# Autodesk Inventor assembly: sestava tělo estonsko s plechem otočené motory
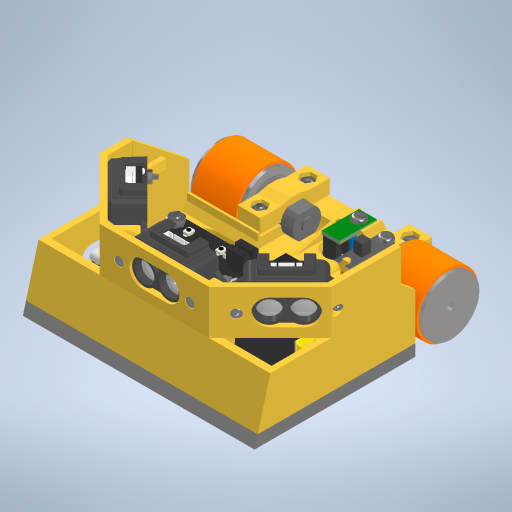
[picture p0: Inventor's stored thumbnail of the model, 512x512]
Saved by Autodesk Inventor 2024 (Build 280153000, 153)
## iProperties
Created: 2023-11-14
Part Number: sestava tělo estonsko s plechem otočené motory
Document SubType Name: Assembly
Designer: Simak
Author: Simak
## Documents named in this file (22)
- C:\Users\Simak\OneDrive\Dokumenty\GitHub\RoboCop\- 3D -\archive\body_v3.0_(Estonsko)\Tělo s plechem\sestava tělo estonsko s plechem otočené motory.iam
- C:\Users\Simak\OneDrive\Dokumenty\GitHub\RoboCop\- 3D -\archive\body_v3.0_(Estonsko)\Tělo s plechem\tělo estonsko s plechem otočené motory.ipt
- C:\Users\Simak\OneDrive\Dokumenty\GitHub\RoboCop\- 3D -\mech._parts\plech.ipt
- C:\Users\Simak\OneDrive\Dokumenty\GitHub\RoboCop\- 3D -\el._parts\sumec_smd.iam
- C:\Users\Simak\OneDrive\Dokumenty\GitHub\RoboCop\- 3D -\archive\TF-Luna_holder_v1\Sestava TF-Luna a držáku.iam
- C:\Users\Simak\OneDrive\Dokumenty\GitHub\RoboCop\- 3D -\el._parts\qre_module.ipt
- C:\Users\Simak\OneDrive\Dokumenty\GitHub\RoboCop\- 3D -\el._parts\switch.ipt
- C:\Users\Simak\OneDrive\Dokumenty\GitHub\RoboCop\- 3D -\el._parts\GA12-N20_Motor.ipt
- C:\Users\Simak\OneDrive\Dokumenty\GitHub\RoboCop\- 3D -\mech._parts\wheel+silicon.ipt
- C:\Users\Simak\OneDrive\Dokumenty\GitHub\RoboCop\- 3D -\mech._parts\motor_C_clamp_nutt_motor_otoceny.ipt
- C:\Users\Simak\OneDrive\Dokumenty\GitHub\RoboCop\- 3D -\screws+nuts\screws\M3_kuzel_torx\torx_socket_countersunk_flat_head_M3x18.ipt
- C:\Users\Simak\OneDrive\Dokumenty\GitHub\RoboCop\- 3D -\screws+nuts\nuts\M3 Nut.ipt
- C:\Users\Simak\OneDrive\Dokumenty\GitHub\RoboCop\- 3D -\screws+nuts\screws\M3_kuzel_torx\torx_socket_countersunk_flat_head_M3x08.ipt
- C:\Users\Simak\OneDrive\Dokumenty\GitHub\RoboCop\- 3D -\screws+nuts\screws\M3_koule_torx\torx_socket_button_head_M3x08.ipt
- C:\Users\Simak\OneDrive\Dokumenty\GitHub\RoboCop\- 3D -\screws+nuts\screws\M3_kuzel_torx\torx_socket_countersunk_flat_head_M3x12.ipt
- C:\Users\Simak\OneDrive\Dokumenty\GitHub\RoboCop\- 3D -\screws+nuts\screws\M3_koule_torx\torx_socket_button_head_M3x10.ipt
- C:\Users\Simak\OneDrive\Dokumenty\GitHub\RoboCop\- 3D -\screws+nuts\screws\M2_valec_imbus\M2 x 0.4mm Thread 16mm LONG SOCKET HEAD CAP SCREW.ipt
- C:\Users\Simak\OneDrive\Dokumenty\GitHub\RoboCop\- 3D -\screws+nuts\screws\M2_valec_imbus\M2 x 0.4mm Thread 12mm LONG SOCKET HEAD CAP SCREW.ipt
- C:\Users\Simak\OneDrive\Dokumenty\GitHub\RoboCop\- 3D -\el._parts\connectors\XT30\XT30_Stecker.ipt
- C:\Users\Simak\OneDrive\Dokumenty\GitHub\RoboCop\- 3D -\screws+nuts\nuts\M2 x 0.4mm Thread HEX NUT.ipt
- C:\Users\Simak\OneDrive\Dokumenty\GitHub\RoboCop\- 3D -\mech._parts\oddělovací plocha.ipt
- C:\Users\Simak\OneDrive\Dokumenty\GitHub\RoboCop\- 3D -\archive\body_v3.0_(Estonsko)\Tělo s plechem\kryt.ipt
## Components (51 placed, 21 different names)
1. tělo estonsko s plechem otočené motory:1 — Proti sobě:1, Stejný směr:1, Stejný směr:2, Proti sobě:2, Vložit:1, Vložit:2, Proti sobě:3, Proti sobě:4, Stejný směr:3, Vložit:3, Proti sobě:5, Proti sobě:6, Proti sobě:7, Proti sobě:8, Proti sobě:10, Proti sobě:11, Proti sobě:12, Proti sobě:13, Proti sobě:14, Proti sobě:15, Stejný směr:4, Stejný směr:5, Proti sobě:19, Vložit:4, Proti sobě:21, Vložit:5, Vložit:8, Vložit:9, Proti sobě:28, Proti sobě:39, Proti sobě:40, Vložit:27, Vložit:28, Proti sobě:41, Proti sobě:42, Vložit:34, Proti sobě:45, Proti sobě:47, Proti sobě:48, Proti sobě:49, Stejný směr:6
2. plech:1 — Proti sobě:1, Stejný směr:1, Stejný směr:2, Vložit:6, Vložit:7, Vložit:11, Vložit:12, Vložit:13, Vložit:14, Proti sobě:46, Vložit:35
3. sumec_smd:1 [sub-assembly] — Proti sobě:2, Vložit:1, Vložit:2, Proti sobě:34, Proti sobě:35, Proti sobě:36, Vložit:23, Vložit:24, Vložit:25, Vložit:26
4. Sestava TF-Luna a držáku:1 [sub-assembly] — Proti sobě:3, Proti sobě:4, Stejný směr:3, Proti sobě:30, Proti sobě:31, Proti sobě:32, Proti sobě:33, Vložit:15, Vložit:16, Vložit:17, Vložit:18, Vložit:19, Vložit:20, Proti sobě:44, Vložit:29, Vložit:30, Vložit:31, Vložit:32, Vložit:33
5. qre_module:1 — Vložit:3, Proti sobě:5, Vložit:10
6. switch:1 — Proti sobě:6, Proti sobě:7, Proti sobě:8, Proti sobě:29
7. GA12-N20_Motor:1 — Proti sobě:13, Proti sobě:14, Proti sobě:15, Proti sobě:17, Proti sobě:20
8. GA12-N20_Motor:2 — Proti sobě:10, Proti sobě:11, Proti sobě:12, Proti sobě:16, Proti sobě:18
9. wheel+silicon:1 — Stejný směr:5, Proti sobě:17
10. wheel+silicon:2 — Stejný směr:4, Proti sobě:16
11. motor_C_clamp_nutt_motor_otoceny:1 — Proti sobě:18, Proti sobě:19, Vložit:4, Proti sobě:22, Proti sobě:24, Vložit:21, Proti sobě:37
12. motor_C_clamp_nutt_motor_otoceny:2 — Proti sobě:20, Proti sobě:21, Vložit:5, Proti sobě:25, Proti sobě:27, Vložit:22, Proti sobě:38
13. torx_socket_countersunk_flat_head_M3x18:1 — Vložit:7, Proti sobě:23
14. torx_socket_countersunk_flat_head_M3x18:2 — Vložit:6, Proti sobě:26
15. M3 Nut:6 — Proti sobě:25, Proti sobě:26, Proti sobě:27
16. M3 Nut:8 — Proti sobě:22, Proti sobě:23, Proti sobě:24
17. torx_socket_countersunk_flat_head_M3x08:1 — Vložit:9
18. torx_socket_countersunk_flat_head_M3x08:2 — Vložit:8
19. torx_socket_button_head_M3x08:1 — Vložit:10
20. torx_socket_button_head_M3x08:2 — Proti sobě:28, Proti sobě:29
21. torx_socket_countersunk_flat_head_M3x12:1 — Vložit:14
22. torx_socket_countersunk_flat_head_M3x12:2 — Vložit:12
23. torx_socket_countersunk_flat_head_M3x12:3 — Vložit:13
24. torx_socket_countersunk_flat_head_M3x12:4 — Vložit:11
25. torx_socket_button_head_M3x10:1 — Proti sobě:31, Proti sobě:32
26. torx_socket_button_head_M3x10:2 — Proti sobě:30, Proti sobě:33
27. M2 x 0.4mm Thread 16mm LONG SOCKET HEAD CAP SCREW:1 — Vložit:18
28. M2 x 0.4mm Thread 16mm LONG SOCKET HEAD CAP SCREW:2 — Vložit:17
29. M2 x 0.4mm Thread 16mm LONG SOCKET HEAD CAP SCREW:3 — Vložit:16
30. M2 x 0.4mm Thread 16mm LONG SOCKET HEAD CAP SCREW:4 — Vložit:15
31. M2 x 0.4mm Thread 12mm LONG SOCKET HEAD CAP SCREW:1 — Vložit:20
32. M2 x 0.4mm Thread 12mm LONG SOCKET HEAD CAP SCREW:2 — Vložit:19, Proti sobě:43
33. XT30_Stecker:1 — Proti sobě:34, Proti sobě:35, Proti sobě:36
34. M3 Nut:9 — Vložit:24
35. M3 Nut:10 — Vložit:23
36. M3 Nut:11 — Proti sobě:39, Proti sobě:40
37. M3 Nut:12 — Vložit:21, Proti sobě:37
38. M3 Nut:13 — Vložit:22, Proti sobě:38
39. M3 Nut:14 — Vložit:25
40. M3 Nut:15 — Vložit:26
41. M3 Nut:16 — Vložit:28, Proti sobě:41
42. M3 Nut:17 — Vložit:27, Proti sobě:42
43. M2 x 0.4mm Thread HEX NUT:1 — Vložit:31
44. M2 x 0.4mm Thread HEX NUT:2 — Vložit:30
45. M2 x 0.4mm Thread HEX NUT:3 — Vložit:33
46. M2 x 0.4mm Thread HEX NUT:4 — Vložit:32
47. M2 x 0.4mm Thread HEX NUT:5 — Vložit:29
48. M2 x 0.4mm Thread HEX NUT:6 — Proti sobě:43, Proti sobě:44
49. M3 Nut:18 — Vložit:34, Proti sobě:45
50. oddělovací plocha:1 — Proti sobě:46, Vložit:35, Proti sobě:47
51. kryt:1 — Proti sobě:48, Proti sobě:49, Stejný směr:6
## Relationships (89: Mate 48, Insert 35, Flush 6)
- Proti sobě:1 [Mate]: tělo estonsko s plechem otočené motory:1 ↔ plech:1
- Stejný směr:1 [Flush]: tělo estonsko s plechem otočené motory:1 ↔ plech:1
- Stejný směr:2 [Flush]: tělo estonsko s plechem otočené motory:1 ↔ plech:1
- Proti sobě:2 [Mate]: tělo estonsko s plechem otočené motory:1 ↔ sumec_smd:1
- Vložit:1 [Insert]: tělo estonsko s plechem otočené motory:1 ↔ sumec_smd:1
- Vložit:2 [Insert]: tělo estonsko s plechem otočené motory:1 ↔ sumec_smd:1
- Proti sobě:3 [Mate]: tělo estonsko s plechem otočené motory:1 ↔ Sestava TF-Luna a držáku:1
- Proti sobě:4 [Mate]: tělo estonsko s plechem otočené motory:1 ↔ Sestava TF-Luna a držáku:1
- Stejný směr:3 [Flush]: tělo estonsko s plechem otočené motory:1 ↔ Sestava TF-Luna a držáku:1
- Vložit:3 [Insert]: tělo estonsko s plechem otočené motory:1 ↔ qre_module:1
- Proti sobě:5 [Mate]: tělo estonsko s plechem otočené motory:1 ↔ qre_module:1
- Proti sobě:6 [Mate]: tělo estonsko s plechem otočené motory:1 ↔ switch:1
- Proti sobě:7 [Mate]: tělo estonsko s plechem otočené motory:1 ↔ switch:1
- Proti sobě:8 [Mate]: tělo estonsko s plechem otočené motory:1 ↔ switch:1
- Proti sobě:10 [Mate]: tělo estonsko s plechem otočené motory:1 ↔ GA12-N20_Motor:2
- Proti sobě:11 [Mate]: tělo estonsko s plechem otočené motory:1 ↔ GA12-N20_Motor:2
- Proti sobě:12 [Mate]: tělo estonsko s plechem otočené motory:1 ↔ GA12-N20_Motor:2
- Proti sobě:13 [Mate]: tělo estonsko s plechem otočené motory:1 ↔ GA12-N20_Motor:1
- Proti sobě:14 [Mate]: tělo estonsko s plechem otočené motory:1 ↔ GA12-N20_Motor:1
- Proti sobě:15 [Mate]: tělo estonsko s plechem otočené motory:1 ↔ GA12-N20_Motor:1
- Stejný směr:4 [Flush]: tělo estonsko s plechem otočené motory:1 ↔ wheel+silicon:2
- Proti sobě:16 [Mate]: GA12-N20_Motor:2 ↔ wheel+silicon:2
- Stejný směr:5 [Flush]: tělo estonsko s plechem otočené motory:1 ↔ wheel+silicon:1
- Proti sobě:17 [Mate]: GA12-N20_Motor:1 ↔ wheel+silicon:1
- Proti sobě:18 [Mate]: GA12-N20_Motor:2 ↔ motor_C_clamp_nutt_motor_otoceny:1
- Proti sobě:19 [Mate]: tělo estonsko s plechem otočené motory:1 ↔ motor_C_clamp_nutt_motor_otoceny:1
- Vložit:4 [Insert]: tělo estonsko s plechem otočené motory:1 ↔ motor_C_clamp_nutt_motor_otoceny:1
- Proti sobě:20 [Mate]: GA12-N20_Motor:1 ↔ motor_C_clamp_nutt_motor_otoceny:2
- Proti sobě:21 [Mate]: tělo estonsko s plechem otočené motory:1 ↔ motor_C_clamp_nutt_motor_otoceny:2
- Vložit:5 [Insert]: tělo estonsko s plechem otočené motory:1 ↔ motor_C_clamp_nutt_motor_otoceny:2
- Vložit:6 [Insert]: plech:1 ↔ torx_socket_countersunk_flat_head_M3x18:2
- Vložit:7 [Insert]: plech:1 ↔ torx_socket_countersunk_flat_head_M3x18:1
- Proti sobě:22 [Mate]: motor_C_clamp_nutt_motor_otoceny:1 ↔ M3 Nut:8
- Proti sobě:23 [Mate]: torx_socket_countersunk_flat_head_M3x18:1 ↔ M3 Nut:8
- Proti sobě:24 [Mate]: motor_C_clamp_nutt_motor_otoceny:1 ↔ M3 Nut:8
- Proti sobě:25 [Mate]: motor_C_clamp_nutt_motor_otoceny:2 ↔ M3 Nut:6
- Proti sobě:26 [Mate]: torx_socket_countersunk_flat_head_M3x18:2 ↔ M3 Nut:6
- Proti sobě:27 [Mate]: motor_C_clamp_nutt_motor_otoceny:2 ↔ M3 Nut:6
- Vložit:8 [Insert]: tělo estonsko s plechem otočené motory:1 ↔ torx_socket_countersunk_flat_head_M3x08:2
- Vložit:9 [Insert]: tělo estonsko s plechem otočené motory:1 ↔ torx_socket_countersunk_flat_head_M3x08:1
- Vložit:10 [Insert]: qre_module:1 ↔ torx_socket_button_head_M3x08:1
- Proti sobě:28 [Mate]: tělo estonsko s plechem otočené motory:1 ↔ torx_socket_button_head_M3x08:2
- Proti sobě:29 [Mate]: switch:1 ↔ torx_socket_button_head_M3x08:2
- Vložit:11 [Insert]: plech:1 ↔ torx_socket_countersunk_flat_head_M3x12:4
- Vložit:12 [Insert]: plech:1 ↔ torx_socket_countersunk_flat_head_M3x12:2
- Vložit:13 [Insert]: plech:1 ↔ torx_socket_countersunk_flat_head_M3x12:3
- Vložit:14 [Insert]: plech:1 ↔ torx_socket_countersunk_flat_head_M3x12:1
- Proti sobě:30 [Mate]: Sestava TF-Luna a držáku:1 ↔ torx_socket_button_head_M3x10:2
- Proti sobě:31 [Mate]: Sestava TF-Luna a držáku:1 ↔ torx_socket_button_head_M3x10:1
- Proti sobě:32 [Mate]: Sestava TF-Luna a držáku:1 ↔ torx_socket_button_head_M3x10:1
- Proti sobě:33 [Mate]: Sestava TF-Luna a držáku:1 ↔ torx_socket_button_head_M3x10:2
- Vložit:15 [Insert]: Sestava TF-Luna a držáku:1 ↔ M2 x 0.4mm Thread 16mm LONG SOCKET HEAD CAP SCREW:4
- Vložit:16 [Insert]: Sestava TF-Luna a držáku:1 ↔ M2 x 0.4mm Thread 16mm LONG SOCKET HEAD CAP SCREW:3
- Vložit:17 [Insert]: Sestava TF-Luna a držáku:1 ↔ M2 x 0.4mm Thread 16mm LONG SOCKET HEAD CAP SCREW:2
- Vložit:18 [Insert]: Sestava TF-Luna a držáku:1 ↔ M2 x 0.4mm Thread 16mm LONG SOCKET HEAD CAP SCREW:1
- Vložit:19 [Insert]: Sestava TF-Luna a držáku:1 ↔ M2 x 0.4mm Thread 12mm LONG SOCKET HEAD CAP SCREW:2
- Vložit:20 [Insert]: Sestava TF-Luna a držáku:1 ↔ M2 x 0.4mm Thread 12mm LONG SOCKET HEAD CAP SCREW:1
- Proti sobě:34 [Mate]: sumec_smd:1 ↔ XT30_Stecker:1
- Proti sobě:35 [Mate]: sumec_smd:1 ↔ XT30_Stecker:1
- Proti sobě:36 [Mate]: sumec_smd:1 ↔ XT30_Stecker:1
- Vložit:21 [Insert]: motor_C_clamp_nutt_motor_otoceny:1 ↔ M3 Nut:12
- Proti sobě:37 [Mate]: motor_C_clamp_nutt_motor_otoceny:1 ↔ M3 Nut:12
- Vložit:22 [Insert]: motor_C_clamp_nutt_motor_otoceny:2 ↔ M3 Nut:13
- Proti sobě:38 [Mate]: motor_C_clamp_nutt_motor_otoceny:2 ↔ M3 Nut:13
- Proti sobě:39 [Mate]: tělo estonsko s plechem otočené motory:1 ↔ M3 Nut:11
- Proti sobě:40 [Mate]: tělo estonsko s plechem otočené motory:1 ↔ M3 Nut:11
- Vložit:23 [Insert]: sumec_smd:1 ↔ M3 Nut:10
- Vložit:24 [Insert]: sumec_smd:1 ↔ M3 Nut:9
- Vložit:25 [Insert]: sumec_smd:1 ↔ M3 Nut:14
- Vložit:26 [Insert]: sumec_smd:1 ↔ M3 Nut:15
- Vložit:27 [Insert]: tělo estonsko s plechem otočené motory:1 ↔ M3 Nut:17
- Vložit:28 [Insert]: tělo estonsko s plechem otočené motory:1 ↔ M3 Nut:16
- Proti sobě:41 [Mate]: tělo estonsko s plechem otočené motory:1 ↔ M3 Nut:16
- Proti sobě:42 [Mate]: tělo estonsko s plechem otočené motory:1 ↔ M3 Nut:17
- Proti sobě:43 [Mate]: M2 x 0.4mm Thread 12mm LONG SOCKET HEAD CAP SCREW:2 ↔ M2 x 0.4mm Thread HEX NUT:6
- Proti sobě:44 [Mate]: Sestava TF-Luna a držáku:1 ↔ M2 x 0.4mm Thread HEX NUT:6
- Vložit:29 [Insert]: Sestava TF-Luna a držáku:1 ↔ M2 x 0.4mm Thread HEX NUT:5
- Vložit:30 [Insert]: Sestava TF-Luna a držáku:1 ↔ M2 x 0.4mm Thread HEX NUT:2
- Vložit:31 [Insert]: Sestava TF-Luna a držáku:1 ↔ M2 x 0.4mm Thread HEX NUT:1
- Vložit:32 [Insert]: Sestava TF-Luna a držáku:1 ↔ M2 x 0.4mm Thread HEX NUT:4
- Vložit:33 [Insert]: Sestava TF-Luna a držáku:1 ↔ M2 x 0.4mm Thread HEX NUT:3
- Vložit:34 [Insert]: tělo estonsko s plechem otočené motory:1 ↔ M3 Nut:18
- Proti sobě:45 [Mate]: tělo estonsko s plechem otočené motory:1 ↔ M3 Nut:18
- Proti sobě:46 [Mate]: plech:1 ↔ oddělovací plocha:1
- Vložit:35 [Insert]: plech:1 ↔ oddělovací plocha:1
- Proti sobě:47 [Mate]: tělo estonsko s plechem otočené motory:1 ↔ oddělovací plocha:1
- Proti sobě:48 [Mate]: tělo estonsko s plechem otočené motory:1 ↔ kryt:1
- Proti sobě:49 [Mate]: tělo estonsko s plechem otočené motory:1 ↔ kryt:1
- Stejný směr:6 [Flush]: tělo estonsko s plechem otočené motory:1 ↔ kryt:1
